# Autodesk Inventor assembly: PotAttachmentB10R
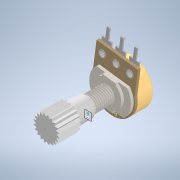
[picture p0: Inventor's stored thumbnail of the model, 180x180]
Saved by Autodesk Inventor 2022 (Build 260153000, 153)
## iProperties
Created: 2021-12-04
Part Number: PotAttachmentB10R
Document SubType Name: Assembly
Designer: teh18
Author: teh18
## iProperties of the stored document Pin2.ipt
Created: 2021-12-04
Part Number: Pin2
Material: Steel
Document SubType Name: Modeling
Designer: teh18
Density: 7.85 g/cm^3
Appearance: Default
Author: teh18
## iProperties of the stored document ScrewBase.ipt
Created: 2021-12-04
Part Number: ScrewBase
Material: Steel
Document SubType Name: Modeling
Designer: teh18
Density: 7.85 g/cm^3
Appearance: Default
Author: teh18
## iProperties of the stored document Pin3.ipt
Created: 2021-12-04
Part Number: Pin3
Material: Steel
Document SubType Name: Modeling
Designer: teh18
Density: 7.85 g/cm^3
Appearance: Default
Author: teh18
## iProperties of the stored document Board.ipt
Created: 2021-12-04
Part Number: Board
Material: Steel
Document SubType Name: Modeling
Designer: teh18
Density: 7.85 g/cm^3
Appearance: Default
Author: teh18
## iProperties of the stored document Casing.ipt
Created: 2021-12-04
Part Number: Casing
Material: Steel
Document SubType Name: Modeling
Designer: teh18
Density: 7.85 g/cm^3
Appearance: Default
Author: teh18
## iProperties of the stored document Pin1.ipt
Created: 2021-12-04
Part Number: Pin1
Material: Steel
Document SubType Name: Modeling
Designer: teh18
Density: 7.85 g/cm^3
Appearance: Default
Author: teh18
## iProperties of the stored document PotentiometerB10K.iam
Created: 2020-08-30
Part Number: PotentiometerB10K
Document SubType Name: Assembly
Designer: teh18
Title: D:/OneDrive/Projetos/Yoke FS/V4/PotentiometerToGrabCad/PotentiometerB10K.step
Sending System: Autodesk Translation Framework v9.3.0.1241
Preprocessor: ST-DEVELOPER v18.1
## iProperties of the stored document Shaft.ipt
Created: 2021-12-04
Part Number: Shaft
Material: Steel
Document SubType Name: Modeling
Designer: teh18
Density: 7.85 g/cm^3
Appearance: Default
Author: teh18
## Documents named in this file (11)
- **C:\Users\teh18\Documents\GitHub\r68-bve-mascon\handle-base\PotAttachmentB10R.iam*LocalDocs*xAaaaahdaAaaaaaaaAaaaakmp2a*Pin2.ipt
- **C:\Users\teh18\Documents\GitHub\r68-bve-mascon\handle-base\PotAttachmentB10R.iam*LocalDocs*xAaaaafdaAaaaaaaaAaaaabsy2h*ScrewBase.ipt
- **C:\Users\teh18\Documents\GitHub\r68-bve-mascon\handle-base\PotAttachmentB10R.iam*LocalDocs*xAaaaaccaAaaaaaaaAaaaacpbDa*Pin3.ipt
- **C:\Users\teh18\Documents\GitHub\r68-bve-mascon\handle-base\PotAttachmentB10R.iam*LocalDocs*xAaaaagaaAaaaaaaaAaaaqhofNe*Board.ipt
- **C:\Users\teh18\Documents\GitHub\r68-bve-mascon\handle-base\PotAttachmentB10R.iam*LocalDocs*xAaaaqjcaAaaaaaaaAaaaat2iQd*Casing.ipt
- **C:\Users\teh18\Documents\GitHub\r68-bve-mascon\handle-base\PotAttachmentB10R.iam*LocalDocs*xAaaaqfaaAaaaaaaaAaaaaacoRf*Pin1.ipt
- **C:\Users\teh18\Documents\GitHub\r68-bve-mascon\handle-base\PotAttachmentB10R.iam*LocalDocs*xAaaaqhaaAaaaaaaaAaaaaeywQd*PotentiometerB10K.iam
- **C:\Users\teh18\Documents\GitHub\r68-bve-mascon\handle-base\PotAttachmentB10R.iam*LocalDocs*xAaaaqrbaAaaaaaaaAaaaalw5Hb*Shaft.ipt
- C:\Users\teh18\Documents\GitHub\r68-bve-mascon\handle-base\PotAttachmentB10R.iam
- C:\Users\teh18\Documents\GitHub\r68-bve-mascon\handle-base\PotAttachmentB10R.ipt
- C:\Users\teh18\OneDrive\BVE Controller\potentiometer-b10k-1.snapshot.2\PotentiometerB10K.step
## Components (2 placed, 2 different names)
1. PotentiometerB10K:1 [sub-assembly] — Flush:1
2. PotAttachmentB10R:1 — Flush:1
## Relationships (1: Flush 1)
- Flush:1: PotentiometerB10K:1 ↔ PotAttachmentB10R:1
